# Autodesk Inventor assembly: PlacaEnsamble
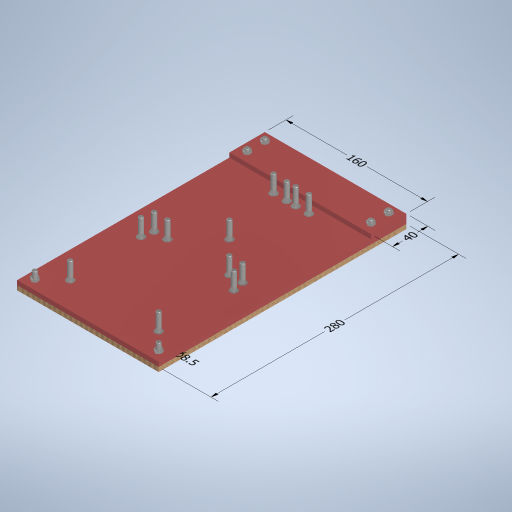
[picture p0: Inventor's stored thumbnail of the model, 512x512]
Saved by Autodesk Inventor 2023.1 (Build 271208000, 208)
## iProperties
Created: 2022-11-01
Part Number: PlacaEnsamble
Document SubType Name: Assembly
Designer: Daniel Peña
Author: Daniel Peña
## Documents named in this file (7)
- C:\Users\danie\Documents\UN\ProyectoRobotica\CAD\PlacaEnsamble\PlacaEnsamble.iam
- C:\Users\danie\Documents\UN\ProyectoRobotica\CAD\V2\GripperV2.iam
- C:\Users\danie\Documents\UN\ProyectoRobotica\CAD\PlacaEnsamble\BaseEnsamble.ipt
- C:\Users\danie\Documents\UN\ProyectoRobotica\CAD\PlacaEnsamble\ReposadorPinzas.ipt
- C:\Users\danie\Documents\Inventor\Content Center Files\R2023\en-US\AS 1420\AS 1420 - 1973 - M5 x 20.ipt
- C:\Users\danie\Documents\UN\ProyectoRobotica\CAD\PlacaEnsamble\BasePiso.ipt
- C:\Users\danie\Documents\Inventor\Content Center Files\R2023\en-US\AS 1112 (2)\AS 1112 - M4  Type 5.ipt
## Components (33 placed, 6 different names)
1. GripperV2:1 [sub-assembly] — Mate:2, Flush:3, Flush:4
2. BaseEnsamble:1 — Flush:1, Flush:2, Mate:1, Flush:3, Flush:4, Flush:5, Insert:1, Insert:2, Insert:3, Insert:4, Insert:5, Insert:6, Insert:7, Insert:8, Insert:9, Insert:10, Insert:11, Insert:12, Insert:13, Flush:7, Flush:8, Mate:3, Insert:20, Insert:21, Insert:22, Insert:23, Insert:24, Insert:25
3. ReposadorPinzas:1 — Flush:1, Flush:2, Mate:1, Mate:2, Flush:5, Insert:26, Insert:27, Insert:28, Insert:29
4. BasePiso:1 — Insert:14, Insert:15, Insert:16, Insert:17, Insert:18, Insert:19, Flush:7, Flush:8, Mate:3
5. AS 1420 - Metric M5 x 20:14 — Insert:15
6. AS 1420 - Metric M5 x 20:15 — Insert:14
7. AS 1420 - Metric M5 x 20:16 — Insert:16
8. AS 1420 - Metric M5 x 20:17 — Insert:17
9. AS 1420 - Metric M5 x 20:18 — Insert:18
10. AS 1420 - Metric M5 x 20:19 — Insert:19
11. AS 1420 - Metric M5 x 20:1 — Insert:4
12. AS 1420 - Metric M5 x 20:2 — Insert:5
13. AS 1420 - Metric M5 x 20:3 — Insert:3
14. AS 1420 - Metric M5 x 20:4 — Insert:1
15. AS 1420 - Metric M5 x 20:5 — Insert:2
16. AS 1420 - Metric M5 x 20:6 — Insert:7
17. AS 1420 - Metric M5 x 20:7 — Insert:8
18. AS 1420 - Metric M5 x 20:8 — Insert:6
19. AS 1420 - Metric M5 x 20:9 — Insert:9
20. AS 1420 - Metric M5 x 20:10 — Insert:10
21. AS 1420 - Metric M5 x 20:11 — Insert:11
22. AS 1420 - Metric M5 x 20:12 — Insert:12
23. AS 1420 - Metric M5 x 20:13 — Insert:13
24. AS 1112 (2) - Metric M4  Type 5:1 — Insert:20
25. AS 1112 (2) - Metric M4  Type 5:2 — Insert:21
26. AS 1112 (2) - Metric M4  Type 5:3 — Insert:22
27. AS 1112 (2) - Metric M4  Type 5:4 — Insert:23
28. AS 1112 (2) - Metric M4  Type 5:5 — Insert:24
29. AS 1112 (2) - Metric M4  Type 5:6 — Insert:25
30. AS 1112 (2) - Metric M4  Type 5:7 — Insert:26
31. AS 1112 (2) - Metric M4  Type 5:8 — Insert:27
32. AS 1112 (2) - Metric M4  Type 5:9 — Insert:28
33. AS 1112 (2) - Metric M4  Type 5:10 — Insert:29
## Relationships (39: Insert 29, Flush 7, Mate 3)
- Flush:1: BaseEnsamble:1 ↔ ReposadorPinzas:1
- Flush:2: BaseEnsamble:1 ↔ ReposadorPinzas:1
- Mate:1: BaseEnsamble:1 ↔ ReposadorPinzas:1
- Mate:2: GripperV2:1 ↔ ReposadorPinzas:1
- Flush:3 (-20 mm): GripperV2:1 ↔ BaseEnsamble:1
- Flush:4 (-20 mm): GripperV2:1 ↔ BaseEnsamble:1
- Flush:5: BaseEnsamble:1 ↔ ReposadorPinzas:1
- Insert:1: BaseEnsamble:1 ↔ AS 1420 - Metric M5 x 20:4
- Insert:2: BaseEnsamble:1 ↔ AS 1420 - Metric M5 x 20:5
- Insert:3: BaseEnsamble:1 ↔ AS 1420 - Metric M5 x 20:3
- Insert:4: BaseEnsamble:1 ↔ AS 1420 - Metric M5 x 20:1
- Insert:5: BaseEnsamble:1 ↔ AS 1420 - Metric M5 x 20:2
- Insert:6: BaseEnsamble:1 ↔ AS 1420 - Metric M5 x 20:8
- Insert:7: BaseEnsamble:1 ↔ AS 1420 - Metric M5 x 20:6
- Insert:8: BaseEnsamble:1 ↔ AS 1420 - Metric M5 x 20:7
- Insert:9: BaseEnsamble:1 ↔ AS 1420 - Metric M5 x 20:9
- Insert:10: BaseEnsamble:1 ↔ AS 1420 - Metric M5 x 20:10
- Insert:11: BaseEnsamble:1 ↔ AS 1420 - Metric M5 x 20:11
- Insert:12: BaseEnsamble:1 ↔ AS 1420 - Metric M5 x 20:12
- Insert:13: BaseEnsamble:1 ↔ AS 1420 - Metric M5 x 20:13
- Insert:14: BasePiso:1 ↔ AS 1420 - Metric M5 x 20:15
- Insert:15: BasePiso:1 ↔ AS 1420 - Metric M5 x 20:14
- Insert:16: BasePiso:1 ↔ AS 1420 - Metric M5 x 20:16
- Insert:17: BasePiso:1 ↔ AS 1420 - Metric M5 x 20:17
- Insert:18: BasePiso:1 ↔ AS 1420 - Metric M5 x 20:18
- Insert:19: BasePiso:1 ↔ AS 1420 - Metric M5 x 20:19
- Flush:7: BaseEnsamble:1 ↔ BasePiso:1
- Flush:8: BaseEnsamble:1 ↔ BasePiso:1
- Mate:3: BaseEnsamble:1 ↔ BasePiso:1
- Insert:20: BaseEnsamble:1 ↔ AS 1112 (2) - Metric M4  Type 5:1
- Insert:21: BaseEnsamble:1 ↔ AS 1112 (2) - Metric M4  Type 5:2
- Insert:22: BaseEnsamble:1 ↔ AS 1112 (2) - Metric M4  Type 5:3
- Insert:23: BaseEnsamble:1 ↔ AS 1112 (2) - Metric M4  Type 5:4
- Insert:24: BaseEnsamble:1 ↔ AS 1112 (2) - Metric M4  Type 5:5
- Insert:25: BaseEnsamble:1 ↔ AS 1112 (2) - Metric M4  Type 5:6
- Insert:26: ReposadorPinzas:1 ↔ AS 1112 (2) - Metric M4  Type 5:7
- Insert:27: ReposadorPinzas:1 ↔ AS 1112 (2) - Metric M4  Type 5:8
- Insert:28: ReposadorPinzas:1 ↔ AS 1112 (2) - Metric M4  Type 5:9
- Insert:29: ReposadorPinzas:1 ↔ AS 1112 (2) - Metric M4  Type 5:10
